# Autodesk Inventor assembly: Stewart-Body-KST215MG
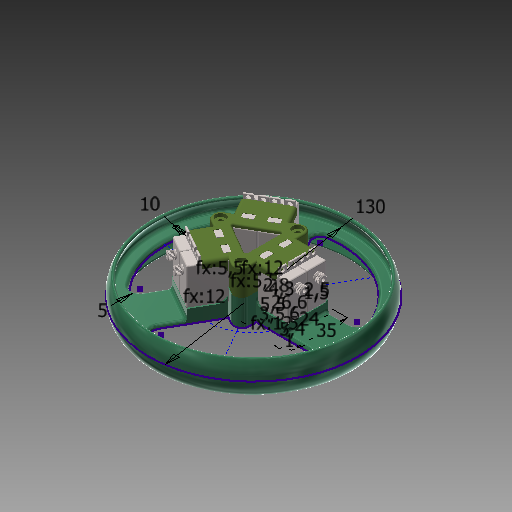
[picture p0: Inventor's stored thumbnail of the model, 512x512]
Saved by Autodesk Inventor 2018.2 (Build 222227000, 227)
## iProperties
Created: 2018-02-25
Part Number: Stewart-Body-KST215MG
Material: Generisch
Document SubType Name: Assembly
Designer: JochenAlt
Author: JochenAlt
## Documents named in this file (4)
- D:\Projects\Donna\CAD\Stewart-Body.iam
- D:\Projects\Donna\CAD\Stewart-Body.ipt
- D:\Projects\Donna\CAD\Servo-KST-DS215MG.ipt
- D:\Projects\Donna\CAD\Ball-Joint-male.ipt
## Components (13 placed, 3 different names)
1. Stewart-Plate:1 — Passend:22, Passend:23, Passend:24, Passend:25, Passend:26, Passend:27, Passend:28, Passend:29, Passend:30, Passend:31, Passend:32, Passend:33, Passend:38, Passend:75, Passend:78, Passend:79, Passend:83, Passend:86, Passend:90, Passend:91, Passend:92, Passend:93, Passend:94, Passend:95, Passend:96, Passend:97, Passend:98, Passend:99, Passend:100, Passend:101, Passend:102, Passend:103
2. Servo-KST-DS215MG:1 — Passend:78, Passend:100, Passend:102
3. Servo-KST-DS215MG:2 — Passend:79, Passend:101, Passend:103
4. Servo-KST-DS215MG:5 — Passend:86, Passend:97, Passend:98
5. Servo-KST-DS215MG:6 — Passend:83, Passend:96, Passend:99
6. ball joint:1 — Passend:22, Passend:28
7. ball joint:2 — Passend:23, Passend:29
8. ball joint:3 — Passend:24, Passend:33
9. ball joint:4 — Passend:25, Passend:32
10. ball joint:5 — Passend:26, Passend:31
11. ball joint:6 — Passend:27, Passend:30
12. Servo-KST-DS215MG:7 — Passend:75, Passend:91, Passend:92, Passend:94
13. Servo-KST-DS215MG:8 — Passend:90, Passend:93, Passend:95
## Relationships (32: Mate 32)
- Passend:22 [Mate]: Stewart-Plate:1 ↔ ball joint:1
- Passend:23 [Mate]: Stewart-Plate:1 ↔ ball joint:2
- Passend:24 [Mate]: Stewart-Plate:1 ↔ ball joint:3
- Passend:25 [Mate]: Stewart-Plate:1 ↔ ball joint:4
- Passend:26 [Mate]: Stewart-Plate:1 ↔ ball joint:5
- Passend:27 [Mate]: Stewart-Plate:1 ↔ ball joint:6
- Passend:28 [Mate]: Stewart-Plate:1 ↔ ball joint:1
- Passend:29 [Mate]: Stewart-Plate:1 ↔ ball joint:2
- Passend:30 [Mate]: Stewart-Plate:1 ↔ ball joint:6
- Passend:31 [Mate]: Stewart-Plate:1 ↔ ball joint:5
- Passend:32 [Mate]: Stewart-Plate:1 ↔ ball joint:4
- Passend:33 [Mate]: Stewart-Plate:1 ↔ ball joint:3
- Passend:38 [Mate]: Stewart-Plate:1
- Passend:75 [Mate]: Stewart-Plate:1 ↔ Servo-KST-DS215MG:7
- Passend:78 [Mate]: Stewart-Plate:1 ↔ Servo-KST-DS215MG:1
- Passend:79 [Mate]: Stewart-Plate:1 ↔ Servo-KST-DS215MG:2
- Passend:83 [Mate]: Stewart-Plate:1 ↔ Servo-KST-DS215MG:6
- Passend:86 [Mate]: Stewart-Plate:1 ↔ Servo-KST-DS215MG:5
- Passend:90 [Mate]: Stewart-Plate:1 ↔ Servo-KST-DS215MG:8
- Passend:91 [Mate]: Stewart-Plate:1 ↔ Servo-KST-DS215MG:7
- Passend:92 [Mate]: Stewart-Plate:1 ↔ Servo-KST-DS215MG:7
- Passend:93 [Mate]: Stewart-Plate:1 ↔ Servo-KST-DS215MG:8
- Passend:94 [Mate]: Stewart-Plate:1 ↔ Servo-KST-DS215MG:7
- Passend:95 [Mate]: Stewart-Plate:1 ↔ Servo-KST-DS215MG:8
- Passend:96 [Mate]: Stewart-Plate:1 ↔ Servo-KST-DS215MG:6
- Passend:97 [Mate]: Stewart-Plate:1 ↔ Servo-KST-DS215MG:5
- Passend:98 [Mate]: Stewart-Plate:1 ↔ Servo-KST-DS215MG:5
- Passend:99 [Mate]: Stewart-Plate:1 ↔ Servo-KST-DS215MG:6
- Passend:100 [Mate]: Stewart-Plate:1 ↔ Servo-KST-DS215MG:1
- Passend:101 [Mate]: Stewart-Plate:1 ↔ Servo-KST-DS215MG:2
- Passend:102 [Mate]: Stewart-Plate:1 ↔ Servo-KST-DS215MG:1
- Passend:103 [Mate]: Stewart-Plate:1 ↔ Servo-KST-DS215MG:2
